# Autodesk Inventor assembly: BandaTrans2
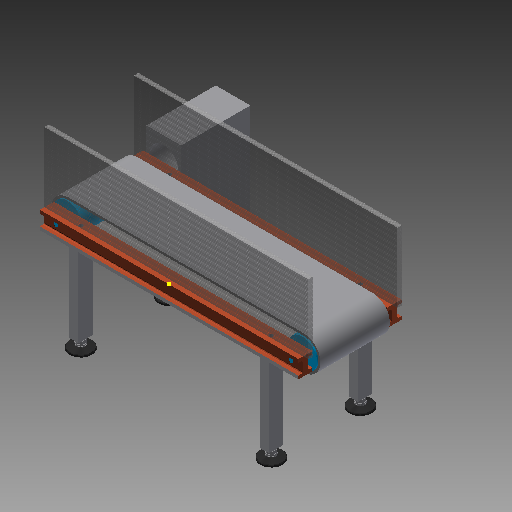
[picture p0: Inventor's stored thumbnail of the model, 512x512]
Saved by Autodesk Inventor 2019 (Build 230136000, 136)
## iProperties
Created: 2019-03-24
Part Number: BandaTrans2
Document SubType Name: Assembly
Designer: felix
Mass: 7303.81 g
Surface Area: 13100.5 cm^2
Volume: 7303.81 cm^3
Density: 1 g/cm^3
Author: felix
## Documents named in this file (7)
- D:\Documents\Inventor\Content Center Files\BandaTrans2.iam
- D:\Documents\Inventor\Content Center Files\Rodo.ipt
- D:\Documents\Inventor\banda1.ipt
- D:\Documents\Inventor\Content Center Files\BarraEx.ipt
- D:\Documents\Inventor\Content Center Files\carril4.ipt
- D:\Downloads\Assembly v7\Leveling leg M10 v3.iam
- D:\Documents\Inventor\Content Center Files\stand2.ipt
## Components (12 placed, 6 different names)
1. Rodo:1 — Mate:21, Mate:22, Mate:24, Mate:27, Mate:30
2. Rodo:2 — Mate:23, Mate:25, Mate:26, Mate:28
3. banda1:1 — Mate:21, Mate:28, Mate:30
4. BarraEx:1 — Mate:22, Mate:23, Mate:24, Mate:31, Flush:1, Flush:3, Rigid:2, Rigid:3
5. BarraEx:2 — Mate:25, Mate:26, Mate:27, Mate:32, Flush:2, Flush:4, Rigid:1, Rigid:4
6. carril4:1 — Mate:31, Flush:1, Flush:3
7. carril4:2 — Mate:32, Flush:2, Flush:4
8. Leveling leg M10 v3:1 [sub-assembly] — Rigid:1
9. Leveling leg M10 v3:2 [sub-assembly] — Rigid:2
10. Leveling leg M10 v3:3 [sub-assembly] — Rigid:4
11. Leveling leg M10 v3:4 [sub-assembly] — Rigid:3
12. stand2:1 — Flush:5, Flush:6, Mate:33
## Relationships (22: Mate 12, Flush 6, WeldJoint 4)
- Mate:21: Rodo:1 ↔ banda1:1
- Mate:22: Rodo:1 ↔ BarraEx:1
- Mate:23: Rodo:2 ↔ BarraEx:1
- Mate:24: Rodo:1 ↔ BarraEx:1
- Mate:25: Rodo:2 ↔ BarraEx:2
- Mate:26: Rodo:2 ↔ BarraEx:2
- Mate:27: Rodo:1 ↔ BarraEx:2
- Mate:28: Rodo:2 ↔ banda1:1
- Mate:30 (2.5 mm): Rodo:1 ↔ banda1:1
- Mate:31: BarraEx:1 ↔ carril4:1
- Mate:32: BarraEx:2 ↔ carril4:2
- Flush:1: BarraEx:1 ↔ carril4:1
- Flush:2: BarraEx:2 ↔ carril4:2
- Flush:3 (10 mm): BarraEx:1 ↔ carril4:1
- Flush:4 (10 mm): BarraEx:2 ↔ carril4:2
- Rigid:1 [WeldJoint] (15 mm): BarraEx:2 ↔ Leveling leg M10 v3:1
- Rigid:2 [WeldJoint] (15 mm): BarraEx:1 ↔ Leveling leg M10 v3:2
- Rigid:3 [WeldJoint] (15 mm): BarraEx:1 ↔ Leveling leg M10 v3:4
- Rigid:4 [WeldJoint] (15 mm): BarraEx:2 ↔ Leveling leg M10 v3:3
- Flush:5 (-547 mm): stand2:1
- Flush:6 (-680 mm): stand2:1
- Mate:33 (-319 mm): stand2:1
